# Autodesk Inventor assembly: 217-2778-001 Rev2_NCQ8A075-050M
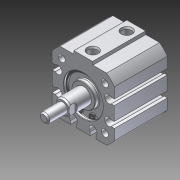
[picture p0: Inventor's stored thumbnail of the model, 180x180]
Saved by Autodesk Inventor 2014 SP1 (Build 180222100, 222)
## iProperties
Created: 2014-01-04
Part Number: 217-2778-001 Rev2_NCQ8A075-050M
Document SubType Name: Assembly
Designer: Moses
Mass: 67.4629 g
Surface Area: 115.13 cm^2
Volume: 19.858 cm^3
Density: 3.39727 g/cm^3
Author: Moses
## Documents named in this file (4)
- C:\Users\Moses\Documents\GitHub\2014buildCAD\chassisdrivetrain\gearbot\217-3433 (3 CIM Gearbox - WC)\217-2778-001 Rev2_NCQ8A075-050M.iam
- C:\Users\Moses\Documents\GitHub\2014buildCAD\chassisdrivetrain\gearbot\217-3433 (3 CIM Gearbox - WC)\217-2778-NCQ8A075-050M_NCQ8 Tube_075A.ipt
- C:\Users\Moses\Documents\GitHub\2014buildCAD\chassisdrivetrain\gearbot\217-3433 (3 CIM Gearbox - WC)\217-2778-NCQ8A075-050M_NCQ8 Rod_075M.ipt
- C:\Users\Moses\Documents\GitHub\2014buildCAD\chassisdrivetrain\gearbot\217-3433 (3 CIM Gearbox - WC)\217-2778-NCQ8A075-050M_Snap Ring_075.ipt
## Components (3 placed, 3 different names)
1. 217-2778-NCQ8A075-050M_NCQ8 Tube_075A_79 — Mate:1, Flush:1, Mate:2
2. 217-2778-NCQ8A075-050M_NCQ8 Rod_075M_80 — Mate:1, Flush:1, Mate:3
3. 217-2778-NCQ8A075-050M_Snap Ring_075_81 — Mate:2, Mate:3
## Relationships (4: Mate 3, Flush 1)
- Mate:1: 217-2778-NCQ8A075-050M_NCQ8 Tube_075A_79 ↔ 217-2778-NCQ8A075-050M_NCQ8 Rod_075M_80
- Flush:1 (-20.0981 mm): 217-2778-NCQ8A075-050M_NCQ8 Tube_075A_79 ↔ 217-2778-NCQ8A075-050M_NCQ8 Rod_075M_80
- Mate:2: 217-2778-NCQ8A075-050M_NCQ8 Tube_075A_79 ↔ 217-2778-NCQ8A075-050M_Snap Ring_075_81
- Mate:3: 217-2778-NCQ8A075-050M_NCQ8 Rod_075M_80 ↔ 217-2778-NCQ8A075-050M_Snap Ring_075_81
